# Autodesk Inventor assembly: topBottomMirror
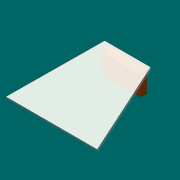
[picture p0: Inventor's stored thumbnail of the model, 180x180]
Saved by Autodesk Inventor 2016 (Build 200138000, 138)
## iProperties
Created: 2015-10-14
Part Number: topBottomMirror
Document SubType Name: Assembly
Designer: Sawaiz
Author: Sawaiz
## Documents named in this file (4)
- C:\Users\sawai\OneDrive\projects\modularRICH\mirror\topBottomMirror.iam
- C:\Users\sawai\OneDrive\projects\modularRICH\mirror\mirrorSupport.ipt
- C:\Users\sawai\OneDrive\projects\modularRICH\mirror\mirrorTopBottom.ipt
- C:\Users\sawai\OneDrive\projects\modularRICH\modularRICH.xlsx
## Components (2 placed, 2 different names)
1. mirrorSupport:1 — Mate:1, Mate:3, Mate:4
2. mirrorTopBottom:1 — Mate:1, Mate:3, Mate:4
## Relationships (3: Mate 3)
- Mate:1: mirrorSupport:1 ↔ mirrorTopBottom:1
- Mate:3 (3.6204 mm): mirrorSupport:1 ↔ mirrorTopBottom:1
- Mate:4: mirrorSupport:1 ↔ mirrorTopBottom:1
## Named parameters: acrylicThickness = 6.35 mm, aerogelThickness = 20 mm, height = 100 mm, width = 100 mm, depth = 100 mm, mirrorAngle = 16 deg, detectorWidth = 52 mm, detectorHeight = 52 mm, mirrorThickness = 3 mm, fresnelThickness = 0.1 mm, grooveDensity = 100, focalLength = 76.2 mm, ior = 1.49, centerThickness = 1.524 mm, fresnelAngle = 90 deg, fresnelEffectiveDiameter = 76.2 mm, mirrorSuppourtWidth = 40 mm
